# Autodesk Inventor assembly: vehicle assembly
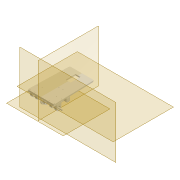
[picture p0: Inventor's stored thumbnail of the model, 180x180]
Saved by Autodesk Inventor 2022 (Build 260153000, 153)
## iProperties
Created: 2024-03-20
Part Number: vehicle assembly
Document SubType Name: Assembly
Designer: david
Author: david
## Documents named in this file (10)
- C:\Users\david\OneDrive\Documents\Inventor\WRO_FE_2024\vehicle assembly.iam
- C:\Users\david\OneDrive\Documents\Inventor\WRO_FE_2024\base plate.ipt
- C:\Users\david\OneDrive\Documents\Inventor\WRO_FE_2024\bearing holder.ipt
- C:\Users\david\OneDrive\Documents\Inventor\WRO_FE_2024\shaft.ipt
- rear shaft.ipt
- C:\Users\david\OneDrive\Documents\Inventor\WRO_FE_2024\dfifferential.ipt
- C:\Users\david\OneDrive\Documents\Inventor\WRO_FE_2024\hobby motor mount.ipt
- C:\Users\david\OneDrive\Documents\Inventor\WRO_FE_2024\driver gear.ipt
- C:\Users\david\OneDrive\Documents\Inventor\WRO_FE_2024\DC Hobby Motor.ipt
- C:\Users\david\OneDrive\Documents\Inventor\WRO_FE_2024\driver gear adapter.ipt
## Components (12 placed, 9 different names)
1. base plate:1 — Flush:1, Flush:2, Flush:3, Insert:1, Insert:2, Insert:3, Insert:4, Insert:5, Insert:6, Insert:7, Insert:8, Insert:22, Insert:23
2. bearing holder:1 — Insert:3, Insert:4
3. bearing holder:2 — Insert:1, Insert:2
4. bearing holder:3 — Insert:5, Insert:6
5. bearing holder:4 — Insert:7, Insert:8, Mate:1
6. right shaft — Mate:1, Angle:1, Insert:20
7. left shaft — Insert:21
8. dfifferential:1 — Flush:4, Tangent:3, Tangent:4, Insert:20, Insert:21, Tangent:5
9. hobby motor mount:1 — Insert:16, Insert:17, Insert:22, Insert:23
10. driver gear:1 — Flush:6, Insert:19, Tangent:5
11. DC Hobby Motor:1 — Insert:16, Insert:17, Insert:18
12. driver gear adapter:1 — Insert:18, Insert:19
## Relationships (29: Insert 16, Flush 5, Angle 4, Tangent 3, Mate 1)
- Flush:1: base plate:1
- Flush:2: base plate:1
- Flush:3: base plate:1
- Insert:1: base plate:1 ↔ bearing holder:2
- Insert:2: base plate:1 ↔ bearing holder:2
- Insert:3: base plate:1 ↔ bearing holder:1
- Insert:4: base plate:1 ↔ bearing holder:1
- Insert:5: base plate:1 ↔ bearing holder:3
- Insert:6: base plate:1 ↔ bearing holder:3
- Insert:7: base plate:1 ↔ bearing holder:4
- Insert:8: base plate:1 ↔ bearing holder:4
- Mate:1: bearing holder:4 ↔ right shaft
- Angle:1 (0 deg): right shaft
- Flush:4: dfifferential:1
- Angle:3 (0 deg)
- Angle:4 (0 deg)
- Tangent:3: dfifferential:1
- Angle:5 (0 deg)
- Tangent:4: dfifferential:1
- Flush:6 (1 mm): driver gear:1
- Insert:16: hobby motor mount:1 ↔ DC Hobby Motor:1
- Insert:17: hobby motor mount:1 ↔ DC Hobby Motor:1
- Insert:18: DC Hobby Motor:1 ↔ driver gear adapter:1
- Insert:19: driver gear:1 ↔ driver gear adapter:1
- Insert:20: right shaft ↔ dfifferential:1
- Insert:21: left shaft ↔ dfifferential:1
- Tangent:5 (2 mm): dfifferential:1 ↔ driver gear:1
- Insert:22: base plate:1 ↔ hobby motor mount:1
- Insert:23: base plate:1 ↔ hobby motor mount:1
